# Autodesk Inventor assembly: Right Drive Assembly
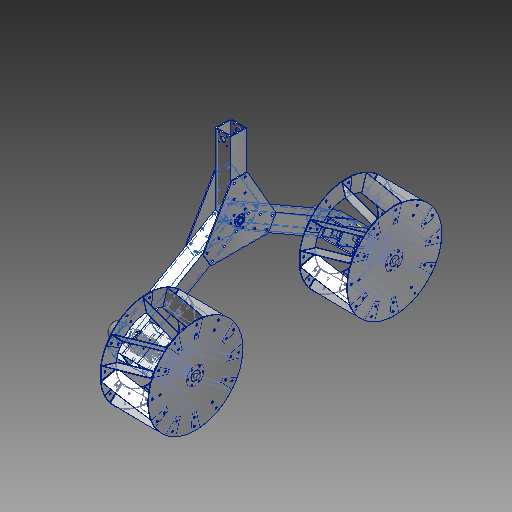
[picture p0: Inventor's stored thumbnail of the model, 512x512]
Saved by Autodesk Inventor 2019 (Build 230136000, 136)
## iProperties
Created: 2018-09-22
Part Number: Right Drive Assembly
Document SubType Name: Assembly
Designer: Adhik
Mass: 6628.82 g
Surface Area: 19020.1 cm^2
Volume: 2342.38 cm^3
Density: 2.82996 g/cm^3
Author: Adhik
## Documents named in this file (5)
- C:\Users\Adhik\Documents\CAD\Julie\Right Drive Assembly.iam
- C:\Users\Adhik\Documents\CAD\Julie\Outer Gusset Plate.ipt
- C:\Users\Adhik\Documents\CAD\Julie\Arm 8 inch.ipt
- C:\Users\Adhik\Documents\CAD\Julie\Arm Bearing.ipt
- C:\Users\Adhik\Documents\CAD\Julie\Drive Arm.iam
## Components (7 placed, 4 different names)
1. Outer Gusset Plate:1 — Mate:25, Mate:27, Mate:28, Insert:1, Mate:31, Mate:32, Mate:33, Mate:34, Mate:35, Mate:36
2. Arm 8 inch:1 — Mate:25, Mate:26, Mate:27, Mate:28, Mate:29, Mate:30
3. Outer Gusset Plate:2 — Mate:26, Mate:29, Mate:30, Insert:2
4. Arm Bearing:1 — Insert:2
5. Arm Bearing:2 — Insert:1
6. Drive Arm:1 [sub-assembly] — Mate:32, Mate:33, Mate:34
7. Drive Arm:2 [sub-assembly] — Mate:31, Mate:35, Mate:36
## Relationships (14: Mate 12, Insert 2)
- Mate:25: Outer Gusset Plate:1 ↔ Arm 8 inch:1
- Mate:26: Arm 8 inch:1 ↔ Outer Gusset Plate:2
- Mate:27: Outer Gusset Plate:1 ↔ Arm 8 inch:1
- Mate:28: Outer Gusset Plate:1 ↔ Arm 8 inch:1
- Mate:29: Arm 8 inch:1 ↔ Outer Gusset Plate:2
- Mate:30: Arm 8 inch:1 ↔ Outer Gusset Plate:2
- Insert:1: Outer Gusset Plate:1 ↔ Arm Bearing:2
- Insert:2: Outer Gusset Plate:2 ↔ Arm Bearing:1
- Mate:31: Outer Gusset Plate:1 ↔ Drive Arm:2
- Mate:32: Outer Gusset Plate:1 ↔ Drive Arm:1
- Mate:33: Outer Gusset Plate:1 ↔ Drive Arm:1
- Mate:34: Outer Gusset Plate:1 ↔ Drive Arm:1
- Mate:35: Outer Gusset Plate:1 ↔ Drive Arm:2
- Mate:36: Outer Gusset Plate:1 ↔ Drive Arm:2
